# Autodesk Inventor assembly: west coast base
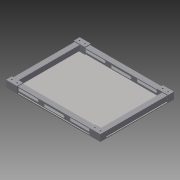
[picture p0: Inventor's stored thumbnail of the model, 180x180]
Saved by Autodesk Inventor 2013 (Build 170138000, 138)
## iProperties
Created: 2014-08-13
Part Number: west coast base
Document SubType Name: Assembly
Designer: kahohbein
Author: kahohbein
## Documents named in this file (5)
- C:\Users\kahohbein\Desktop\west coast base.iam
- C:\Users\kahohbein\Desktop\West Coast Side.ipt
- C:\Users\kahohbein\Desktop\west coast backfront.ipt
- C:\Users\kahohbein\Desktop\west coast corner.ipt
- C:\Users\kahohbein\Desktop\bellypan.ipt
## Components (9 placed, 4 different names)
1. West Coast Side:1 — Mate:2, Flush:1, Flush:2, Mate:3, Mate:9, Mate:12, Mate:16
2. West Coast Side:2 — Mate:2, Flush:1, Flush:2, Flush:3, Mate:4, Mate:7, Mate:11, Flush:4, Mate:15, Flush:6
3. west coast backfront:1 — Mate:11, Flush:4, Mate:12, Mate:13, Mate:14, Mate:17, Mate:18, Flush:5
4. west coast backfront:2 — Flush:3, Mate:3, Mate:4, Mate:5, Mate:6, Mate:8, Mate:10
5. west coast corner:1 — Mate:8, Mate:9, Mate:10
6. west coast corner:2 — Mate:5, Mate:6, Mate:7
7. west coast corner:3 — Mate:14, Mate:15, Mate:17, Mate:19
8. west coast corner:4 — Mate:13, Mate:16, Mate:18
9. bellypan:1 — Mate:19, Flush:5, Flush:6
## Relationships (24: Mate 18, Flush 6)
- Mate:2 (304.8 mm): West Coast Side:1 ↔ West Coast Side:2
- Flush:1: West Coast Side:1 ↔ West Coast Side:2
- Flush:2: West Coast Side:1 ↔ West Coast Side:2
- Flush:3: West Coast Side:2 ↔ west coast backfront:2
- Mate:3: West Coast Side:1 ↔ west coast backfront:2
- Mate:4: West Coast Side:2 ↔ west coast backfront:2
- Mate:5: west coast backfront:2 ↔ west coast corner:2
- Mate:6: west coast backfront:2 ↔ west coast corner:2
- Mate:7: West Coast Side:2 ↔ west coast corner:2
- Mate:8: west coast backfront:2 ↔ west coast corner:1
- Mate:9: West Coast Side:1 ↔ west coast corner:1
- Mate:10: west coast backfront:2 ↔ west coast corner:1
- Mate:11: West Coast Side:2 ↔ west coast backfront:1
- Flush:4: West Coast Side:2 ↔ west coast backfront:1
- Mate:12: West Coast Side:1 ↔ west coast backfront:1
- Mate:13: west coast backfront:1 ↔ west coast corner:4
- Mate:14: west coast backfront:1 ↔ west coast corner:3
- Mate:15: West Coast Side:2 ↔ west coast corner:3
- Mate:16: West Coast Side:1 ↔ west coast corner:4
- Mate:17: west coast backfront:1 ↔ west coast corner:3
- Mate:18: west coast backfront:1 ↔ west coast corner:4
- Mate:19: west coast corner:3 ↔ bellypan:1
- Flush:5: west coast backfront:1 ↔ bellypan:1
- Flush:6: West Coast Side:2 ↔ bellypan:1
